# Autodesk Inventor assembly: Flasche
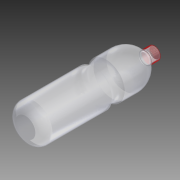
[picture p0: Inventor's stored thumbnail of the model, 180x180]
Saved by Autodesk Inventor 2013 (Build 170138000, 138)
## iProperties
Created: 2012-09-29
Part Number: Flasche
Document SubType Name: Assembly
Designer: fivef
Author: fivef
## Documents named in this file (3)
- D:\Dropbox\My Dropbox\Dokumente\Aktuell\Drinkmixer\Flasche.iam
- D:\Dropbox\My Dropbox\Dokumente\Aktuell\Drinkmixer\Flasche.ipt
- D:\Dropbox\My Dropbox\Dokumente\Aktuell\Drinkmixer\deckel.ipt
## Components (2 placed, 2 different names)
1. Flasche:2 — Einfügen:1
2. deckel:1 — Einfügen:1
## Relationships (1: Insert 1)
- Einfügen:1 [Insert] (15 mm): Flasche:2 ↔ deckel:1
